# Autodesk Inventor assembly: GX12-2 Jack
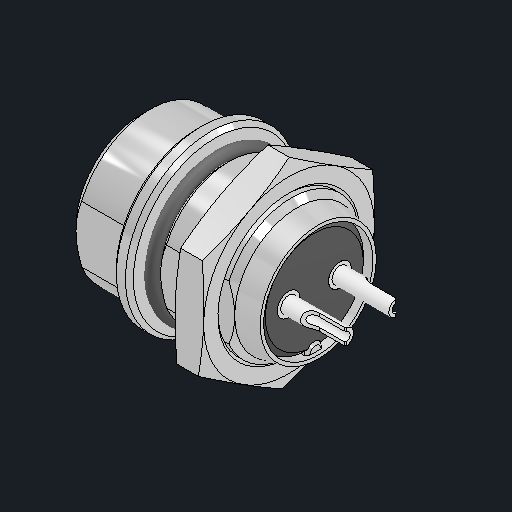
[picture p0: Inventor's stored thumbnail of the model, 512x512]
Saved by Autodesk Inventor 2027.1 (Build 311270010, 270A)
## iProperties
Created: 2024-07-20
Part Number: GX12-2 Jack
Description: FreeCAD Model
Document SubType Name: Assembly
Designer: queezz
Authority: Unknown
Sending System: FreeCAD
Preprocessor: Open CASCADE STEP processor 7.6
Title: Open CASCADE Shape Model
## Documents named in this file (6)
- C:\Users\queezz\Dropbox\Drawings\PIHTI\ContentCenter\Electrics\gx12-aviation-connectors\GX12-2 Jack\GX12-2 Jack.iam
- C:\Users\queezz\Dropbox\Drawings\PIHTI\ContentCenter\Electrics\gx12-aviation-connectors\GX12-2 Jack\GX12-body.ipt
- C:\Users\queezz\Dropbox\Drawings\PIHTI\ContentCenter\Electrics\gx12-aviation-connectors\GX12-2 Jack\GX12-nut.ipt
- C:\Users\queezz\Dropbox\Drawings\PIHTI\ContentCenter\Electrics\gx12-aviation-connectors\GX12-2 Jack\Body002.ipt
- C:\Users\queezz\Dropbox\Drawings\PIHTI\ContentCenter\Electrics\gx12-aviation-connectors\GX12-2 Jack\Body004.ipt
- C:\Users\queezz\Dropbox\Drawings\PIHTI\ContentCenter\Electrics\gx12-aviation-connectors\GX12-2 Jack\Array.iam
## Components (5 placed, 5 different names)
1. 1 — Mate:1
2. 2 — Mate:1
3. 3
4. 4
5. 7 [sub-assembly]
## Relationships (1: Mate 1)
- Mate:1: 1 ↔ 2
